# Autodesk Inventor assembly: New
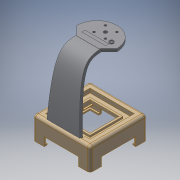
[picture p0: Inventor's stored thumbnail of the model, 180x180]
Saved by Autodesk Inventor 2019 (Build 230136000, 136)
## iProperties
Created: 2017-03-24
Part Number: New
Document SubType Name: Assembly
Designer: Jorian Bruslind
Author: Jorian Bruslind
## Documents named in this file (3)
- C:\Users\Jorian Brusind\Documents\GitHub\PersonalProjects\Automated Terrarium Project\Inventor Files\V2\New assembly.iam
- C:\Users\Jorian Brusind\Documents\GitHub\PersonalProjects\Automated Terrarium Project\Inventor Files\V2\backplaterev2.0.ipt
- C:\Users\Jorian Brusind\Documents\GitHub\PersonalProjects\Automated Terrarium Project\Inventor Files\V2\model for case.ipt
## Components (2 placed, 2 different names)
1. backplaterev2.0:1 — Mate:1, Mate:2
2. model for case:1 — Mate:1, Mate:2
## Relationships (2: Mate 2)
- Mate:1: backplaterev2.0:1 ↔ model for case:1
- Mate:2 (0.7937 mm): backplaterev2.0:1 ↔ model for case:1
